# Autodesk Inventor assembly: main
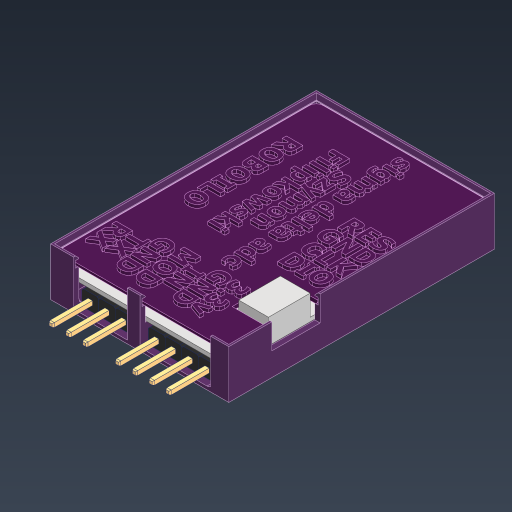
[picture p0: Inventor's stored thumbnail of the model, 512x512]
Saved by Autodesk Inventor 2023 (Build 270158000, 158)
## iProperties
Created: 2025-06-15
Part Number: main
Document SubType Name: Assembly
Designer: szymo
Author: szymo
## Documents named in this file (6)
- D:\tech\konkursy\WETI-2025_26-Szymon_Filipkowski\Inventor-project\main.iam
- D:\tech\konkursy\WETI-2025_26-Szymon_Filipkowski\Inventor-project\adc.ipt
- D:\tech\konkursy\WETI-2025_26-Szymon_Filipkowski\Inventor-project\4x_Male_Pin_2.54_mm.ipt
- D:\tech\konkursy\WETI-2025_26-Szymon_Filipkowski\Inventor-project\3x_Male_Pin_2.54_mm.ipt
- D:\tech\konkursy\WETI-2025_26-Szymon_Filipkowski\Inventor-project\case.ipt
- D:\tech\konkursy\WETI-2025_26-Szymon_Filipkowski\Inventor-project\ceil.ipt
## Components (5 placed, 5 different names)
1. adc:1 — Mate:1, Mate:2, Flush:1, Flush:2, Mate:3, Mate:4, Flush:4
2. 4x_Male_Pin_2.54_mm:1 — Mate:1, Flush:2, Mate:3, Flush:3
3. 3x_Male_Pin_2.54_mm:1 — Mate:2, Flush:1, Mate:4
4. case:1 — Flush:3, Flush:4, Flush:5
5. ceil:1 — Flush:5
## Relationships (9: Flush 5, Mate 4)
- Mate:1 (0.5 mm): adc:1 ↔ 4x_Male_Pin_2.54_mm:1
- Mate:2 (0.5 mm): adc:1 ↔ 3x_Male_Pin_2.54_mm:1
- Flush:1: adc:1 ↔ 3x_Male_Pin_2.54_mm:1
- Flush:2: adc:1 ↔ 4x_Male_Pin_2.54_mm:1
- Mate:3 (2 mm): adc:1 ↔ 4x_Male_Pin_2.54_mm:1
- Mate:4 (2 mm): adc:1 ↔ 3x_Male_Pin_2.54_mm:1
- Flush:3: 4x_Male_Pin_2.54_mm:1 ↔ case:1
- Flush:4: adc:1 ↔ case:1
- Flush:5: case:1 ↔ ceil:1
